# Autodesk Inventor assembly: 左脚ユニット3
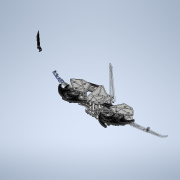
[picture p0: Inventor's stored thumbnail of the model, 180x180]
Saved by Autodesk Inventor 2020 (Build 240168000, 168)
## iProperties
Created: 2019-09-03
Part Number: 左脚ユニット3
Document SubType Name: Assembly
Designer: 雪村
Mass: 943.074 g
Surface Area: 4358.2 cm^2
Volume: 381.562 cm^3
Density: 2.47162 g/cm^3
Author: 雪村
## Documents named in this file (6)
- G:\マイドライブ\かわさき班共有ファイル\02.設計データ\2020年\雪村\2020年機体完成版\部品\左脚ユニット3.iam
- G:\マイドライブ\かわさき班共有ファイル\02.設計データ\2020年\雪村\2020年機体完成版\部品\左脚中間ユニット2.iam
- G:\マイドライブ\かわさき班共有ファイル\02.設計データ\2020年\雪村\2020年機体完成版\部品\左前脚ユニット5.iam
- G:\マイドライブ\かわさき班共有ファイル\02.設計データ\2020年\雪村\2020年機体完成版\部品\左後脚ユニット5.iam
- G:\マイドライブ\かわさき班共有ファイル\02.設計データ\2020年\雪村\2020年機体完成版\部品\平行サスシャフト4.iam
- G:\マイドライブ\かわさき班共有ファイル\02.設計データ\2020年\雪村\2020年機体完成版\パーツ\タミヤダンパー.iam
## Components (6 placed, 5 different names)
1. 左脚中間ユニット2:1 [sub-assembly] — フラッシュ:1, 挿入:3, メイト:1, メイト:2, 挿入:5, 挿入:6
2. 左前脚ユニット5:1 [sub-assembly] — 挿入:1, 挿入:3
3. 左後脚ユニット5:1 [sub-assembly] — 挿入:5, メイト:5
4. 平行サスシャフト4:1 [sub-assembly] — 挿入:1, メイト:1, 挿入:4
5. タミヤダンパー:1 [sub-assembly] — 挿入:4, メイト:2
6. タミヤダンパー:2 [sub-assembly] — メイト:5, 挿入:6
## Relationships (13: Flush 5, Insert 5, Mate 3)
- フラッシュ:1 [Flush] (130 mm): 左脚中間ユニット2:1
- 挿入:1 [Insert]: 左前脚ユニット5:1 ↔ 平行サスシャフト4:1
- 挿入:3 [Insert]: 左脚中間ユニット2:1 ↔ 左前脚ユニット5:1
- メイト:1 [Mate]: 左脚中間ユニット2:1 ↔ 平行サスシャフト4:1
- 挿入:4 [Insert] (10 mm): 平行サスシャフト4:1 ↔ タミヤダンパー:1
- メイト:2 [Mate]: 左脚中間ユニット2:1 ↔ タミヤダンパー:1
- フラッシュ:2 [Flush] (70 mm)
- フラッシュ:3 [Flush] (25 mm)
- フラッシュ:4 [Flush] (-25 mm)
- フラッシュ:5 [Flush] (30 mm)
- 挿入:5 [Insert]: 左脚中間ユニット2:1 ↔ 左後脚ユニット5:1
- メイト:5 [Mate]: 左後脚ユニット5:1 ↔ タミヤダンパー:2
- 挿入:6 [Insert] (4 mm): 左脚中間ユニット2:1 ↔ タミヤダンパー:2
